# Autodesk Inventor assembly: 배터리 홀더
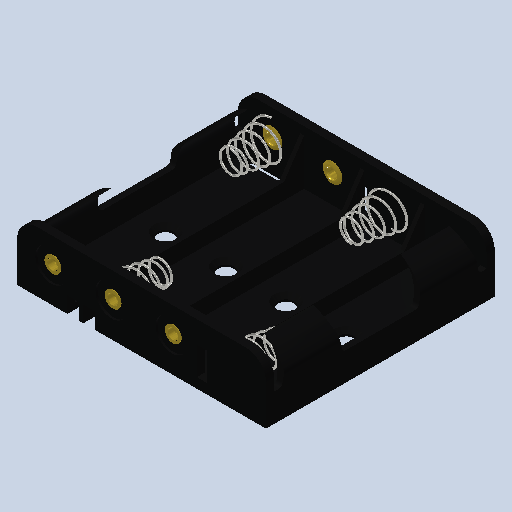
[picture p0: Inventor's stored thumbnail of the model, 512x512]
Saved by Autodesk Inventor 2023.2 (Build 272271030, 271C)
## iProperties
Created: 2018-01-07
Part Number: 배터리 홀더
Document SubType Name: Assembly
Designer: choi jong in
Author: choi jong in
## Documents named in this file (4)
- C:\Users\oktay\Desktop\battery-holder-aasize-1-5v-4-1.snapshot.3\Battery Holder.iam
- C:\Users\oktay\Desktop\battery-holder-aasize-1-5v-4-1.snapshot.3\Battery Holder.ipt
- C:\Users\oktay\Desktop\battery-holder-aasize-1-5v-4-1.snapshot.3\Holder's sub part(copper).ipt
- C:\Users\oktay\Desktop\battery-holder-aasize-1-5v-4-1.snapshot.3\Holder's sub part(spring).ipt
## Components (11 placed, 3 different names)
1. Battery Holder:1 — 플러쉬:1, 메이트:1, 메이트:2, 메이트:3, 메이트:4, 메이트:5, 메이트:6, 메이트:7, 메이트:8, 메이트:9, 메이트:10, 플러쉬:2, 플러쉬:3, 각도:1, 플러쉬:4, 각도:2, 플러쉬:5, 플러쉬:6, 각도:3
2. Holder's sub part(copper):1 — 플러쉬:1
3. Holder's sub part(copper):2 — 메이트:1, 메이트:2, 메이트:12
4. Holder's sub part(copper):3 — 메이트:3, 메이트:4, 메이트:13
5. Holder's sub part(copper):4 — 메이트:9, 메이트:10, 메이트:11
6. Holder's sub part(copper):5 — 메이트:5, 메이트:6, 메이트:14
7. Holder's sub part(copper):6 — 메이트:7, 메이트:8
8. Holder's sub part(spring):1 — 플러쉬:2, 메이트:11, 플러쉬:3
9. Holder's sub part(spring):2 — 메이트:12, 각도:1, 플러쉬:4
10. Holder's sub part(spring):3 — 메이트:13, 각도:2, 플러쉬:5
11. Holder's sub part(spring):4 — 메이트:14, 플러쉬:6, 각도:3
## Relationships (23: Mate 14, Flush 6, Angle 3)
- 플러쉬:1 [Flush]: Battery Holder:1 ↔ Holder's sub part(copper):1
- 메이트:1 [Mate]: Battery Holder:1 ↔ Holder's sub part(copper):2
- 메이트:2 [Mate]: Battery Holder:1 ↔ Holder's sub part(copper):2
- 메이트:3 [Mate]: Battery Holder:1 ↔ Holder's sub part(copper):3
- 메이트:4 [Mate]: Battery Holder:1 ↔ Holder's sub part(copper):3
- 메이트:5 [Mate]: Battery Holder:1 ↔ Holder's sub part(copper):5
- 메이트:6 [Mate]: Battery Holder:1 ↔ Holder's sub part(copper):5
- 메이트:7 [Mate]: Battery Holder:1 ↔ Holder's sub part(copper):6
- 메이트:8 [Mate]: Battery Holder:1 ↔ Holder's sub part(copper):6
- 메이트:9 [Mate]: Battery Holder:1 ↔ Holder's sub part(copper):4
- 메이트:10 [Mate]: Battery Holder:1 ↔ Holder's sub part(copper):4
- 플러쉬:2 [Flush]: Battery Holder:1 ↔ Holder's sub part(spring):1
- 메이트:11 [Mate]: Holder's sub part(copper):4 ↔ Holder's sub part(spring):1
- 플러쉬:3 [Flush]: Battery Holder:1 ↔ Holder's sub part(spring):1
- 메이트:12 [Mate]: Holder's sub part(copper):2 ↔ Holder's sub part(spring):2
- 각도:1 [Angle] (0 deg): Battery Holder:1 ↔ Holder's sub part(spring):2
- 플러쉬:4 [Flush]: Battery Holder:1 ↔ Holder's sub part(spring):2
- 메이트:13 [Mate]: Holder's sub part(copper):3 ↔ Holder's sub part(spring):3
- 각도:2 [Angle] (0 deg): Battery Holder:1 ↔ Holder's sub part(spring):3
- 플러쉬:5 [Flush]: Battery Holder:1 ↔ Holder's sub part(spring):3
- 메이트:14 [Mate]: Holder's sub part(copper):5 ↔ Holder's sub part(spring):4
- 플러쉬:6 [Flush]: Battery Holder:1 ↔ Holder's sub part(spring):4
- 각도:3 [Angle] (0 deg): Battery Holder:1 ↔ Holder's sub part(spring):4
